# Autodesk Inventor assembly: OBG-Mittelschicht
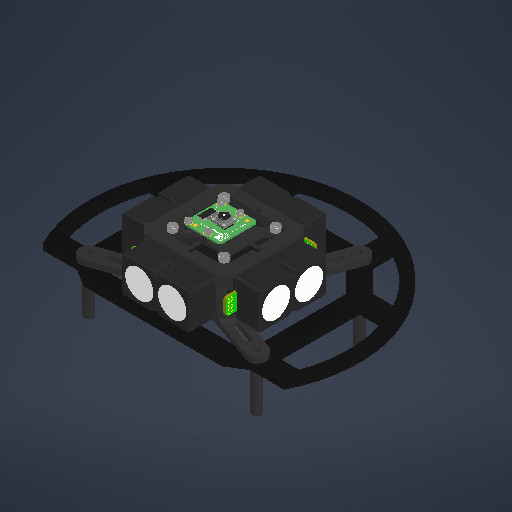
[picture p0: Inventor's stored thumbnail of the model, 512x512]
Saved by Autodesk Inventor 2025.2 (Build 292293000, 293)
## iProperties
Created: 2025-03-28
Part Number: OBG-Mittelschicht
Document SubType Name: Assembly
Designer: Faabs
Author: Faabs
## Documents named in this file (4)
- C:\Users\Faabs\Desktop\TeamFaabs-CAD v2023\OBG\OBG-Mittelschicht.iam
- C:\Users\Faabs\Desktop\TeamFaabs-CAD v2023\OBG\Abstandshalter_Jetson\Abstandshalter_Jetson\Abstandshalter_Jetson.ipt
- C:\Users\Faabs\Desktop\TeamFaabs-CAD v2023\OBG\Plexiglas Ring\Plexiglas Ring\Mittelplatte.ipt
- C:\Users\Faabs\Desktop\TeamFaabs-CAD v2023\UBG\Sensoreinheit\UBG-Sensoreinheit.iam
## Components (6 placed, 3 different names)
1. Mittelplatte:1 — Fluchtend:1, Fluchtend:2, Passend:1, Einfügen:1, Einfügen:2, Einfügen:3, Einfügen:4, Passend:2, Passend:3, Passend:4
2. Abstandshalter_Jetson:1 — Einfügen:4
3. Abstandshalter_Jetson:2 — Einfügen:1
4. Abstandshalter_Jetson:3 — Einfügen:2
5. Abstandshalter_Jetson:4 — Einfügen:3
6. UBG-Sensoreinheit:1 [sub-assembly] — Passend:2, Passend:3, Passend:4
## Relationships (10: Mate 4, Insert 4, Flush 2)
- Fluchtend:1 [Flush]: Mittelplatte:1
- Fluchtend:2 [Flush]: Mittelplatte:1
- Passend:1 [Mate]: Mittelplatte:1
- Einfügen:1 [Insert]: Mittelplatte:1 ↔ Abstandshalter_Jetson:2
- Einfügen:2 [Insert]: Mittelplatte:1 ↔ Abstandshalter_Jetson:3
- Einfügen:3 [Insert]: Mittelplatte:1 ↔ Abstandshalter_Jetson:4
- Einfügen:4 [Insert]: Mittelplatte:1 ↔ Abstandshalter_Jetson:1
- Passend:2 [Mate]: Mittelplatte:1 ↔ UBG-Sensoreinheit:1
- Passend:3 [Mate]: Mittelplatte:1 ↔ UBG-Sensoreinheit:1
- Passend:4 [Mate]: Mittelplatte:1 ↔ UBG-Sensoreinheit:1
